# Autodesk Inventor assembly: Ensamblaje - 2
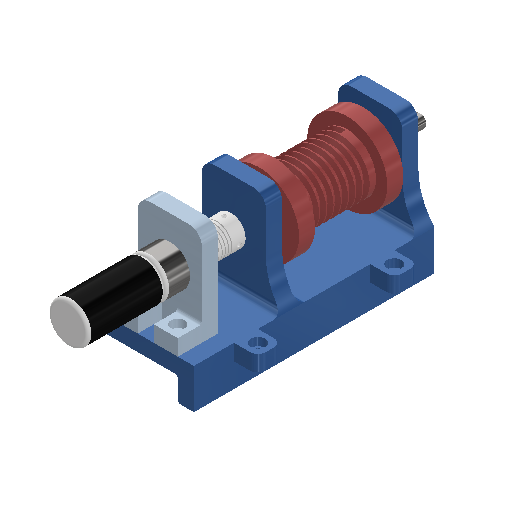
[picture p0: Inventor's stored thumbnail of the model, 512x512]
Saved by Autodesk Inventor 2026.1 (Build 301233000, 233)
## iProperties
Created: 2025-08-27
Part Number: Ensamblaje - 2
Document SubType Name: Assembly
Designer: piero
Author: piero
## Documents named in this file (8)
- D:\Tesis\Modelo 3D\CAD\Ensamblaje - 2.iam
- D:\Tesis\Modelo 3D\CAD\soporte_inferior.ipt
- D:\Tesis\Modelo 3D\CAD\Motor.ipt
- D:\Tesis\Modelo 3D\CAD\acople_suave.ipt
- D:\Tesis\Modelo 3D\CAD\carrete.ipt
- D:\Tesis\Modelo 3D\CAD\perno_pasante.ipt
- D:\Tesis\Modelo 3D\CAD\sujeción motor-acople.ipt
- D:\Tesis\Modelo 3D\CAD\w_608-2rs1.iam
## Components (8 placed, 7 different names)
1. soporte_inferior:1 — Coincidencia:1, Nivelación:1, De rotación:2, De rotación:3, Coincidencia:9, Coincidencia:10
2. Motor:1 — Coincidencia:6, De rotación:1
3. acople_suave:4 — Coincidencia:3, Coincidencia:4, Coincidencia:5
4. carrete:1 — Coincidencia:2
5. perno_pasante:1 — Coincidencia:1, Coincidencia:2, Coincidencia:3, Coincidencia:7, Coincidencia:8
6. sujeción motor-acople:1 — Coincidencia:4, Coincidencia:5, Coincidencia:6, De rotación:1, Coincidencia:9, Coincidencia:10
7. w_608-2rs1:1 [sub-assembly] — Coincidencia:8, De rotación:2
8. w_608-2rs1:2 [sub-assembly] — Coincidencia:7, De rotación:3
## Relationships (14: Mate 10, RevoluteJoint 3, Flush 1)
- Coincidencia:1 [Mate]: soporte_inferior:1 ↔ perno_pasante:1
- Coincidencia:2 [Mate]: carrete:1 ↔ perno_pasante:1
- Coincidencia:3 [Mate]: acople_suave:4 ↔ perno_pasante:1
- Nivelación:1 [Flush] (-15 mm): soporte_inferior:1
- Coincidencia:4 [Mate]: acople_suave:4 ↔ sujeción motor-acople:1
- Coincidencia:5 [Mate]: acople_suave:4 ↔ sujeción motor-acople:1
- Coincidencia:6 [Mate]: Motor:1 ↔ sujeción motor-acople:1
- De rotación:1 [RevoluteJoint]: Motor:1 ↔ sujeción motor-acople:1
- Coincidencia:7 [Mate]: perno_pasante:1 ↔ w_608-2rs1:2
- Coincidencia:8 [Mate]: perno_pasante:1 ↔ w_608-2rs1:1
- De rotación:2 [RevoluteJoint]: soporte_inferior:1 ↔ w_608-2rs1:1
- De rotación:3 [RevoluteJoint]: soporte_inferior:1 ↔ w_608-2rs1:2
- Coincidencia:9 [Mate]: soporte_inferior:1 ↔ sujeción motor-acople:1
- Coincidencia:10 [Mate]: soporte_inferior:1 ↔ sujeción motor-acople:1
